# Autodesk Inventor assembly: Ecran
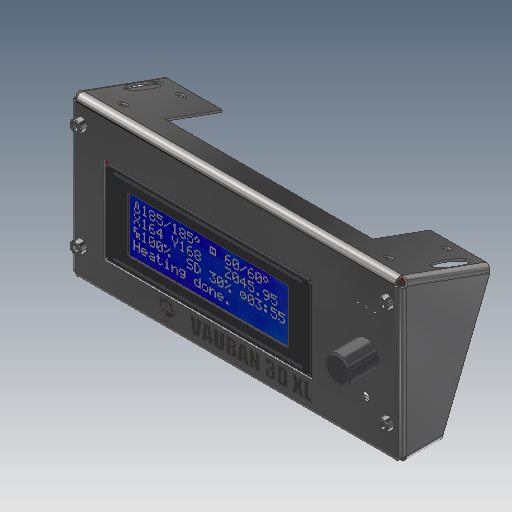
[picture p0: Inventor's stored thumbnail of the model, 512x512]
Saved by Autodesk Inventor 2017 (Build 210142000, 142)
## iProperties
Company: FABLAB Frenchmakers
Part Number: Ecran
Material: Générique
Document SubType Name: Assembly
Designer: FABLAB Frenchmakers
Project: 1420 Vauban 3D XL
Catalog Web Link: http://frenchmakers.com/
Stock Number: 1420-08-00
## Documents named in this file (6)
- W:\Professionnel\Conception FABLAB\1420-Vauban 3D XL\1420-08 Ecran\1420-08-00 Ecran.iam
- W:\Professionnel\Conception FABLAB\1420-Vauban 3D XL\1420-08 Ecran\1420-08-02 Ecran LCD.ipt
- W:\Professionnel\Conception FABLAB\1420-Vauban 3D XL\1420-90 Centre de contenu\fr-FR\ANSI B18.3.1M(1)\ANSI B18.3.1M - M3x0,5 x 20(2).ipt
- W:\Professionnel\Conception FABLAB\1420-Vauban 3D XL\1420-90 Centre de contenu\fr-FR\DIN 934\DIN 934 - M3 x 0,5.ipt
- W:\Professionnel\Conception FABLAB\1420-Vauban 3D XL\1420-08 Ecran\1420-08-01 Boitier tole.ipt
- W:\Professionnel\Conception FABLAB\1420-Vauban 3D XL\1420-08 Ecran\1420-08-03 Carte SD.ipt
## Components (19 placed, 5 different names)
1. 1420-08-02 Ecran LCD:1 — Placage:13, Placage:16, Placage:17, Placage:21, Placage:22, Placage:23, Logement:3, Logement:5, Logement:8, Logement:9, Affleurement:11
2. 1420-08-01 Boitier tole:1 — Placage:14, Affleurement:10, Placage:15, Placage:16, Placage:17, Logement:1, Placage:18, Placage:19, Placage:20, Logement:2, Logement:4, Logement:6, Logement:7, Affleurement:11
3. Vis à tête percée - Métrique M3x0,5 x 20:1 — Affleurement:4, Placage:11, Placage:19
4. Vis à tête percée - Métrique M3x0,5 x 20:2 — Affleurement:4, Affleurement:5, Placage:9, Placage:18
5. Vis à tête percée - Métrique M3x0,5 x 20:3 — Affleurement:5, Affleurement:6, Placage:10, Logement:1
6. Vis à tête percée - Métrique M3x0,5 x 20:4 — Affleurement:6, Placage:12, Placage:20
7. DIN 934 - Remplacé par DIN EN 24032/28673/28674 M3:1 — Affleurement:7, Affleurement:8, Placage:10, Placage:13
8. DIN 934 - Remplacé par DIN EN 24032/28673/28674 M3:2 — Affleurement:8, Affleurement:9, Placage:11
9. DIN 934 - Remplacé par DIN EN 24032/28673/28674 M3:3 — Affleurement:9, Placage:12
10. DIN 934 - Remplacé par DIN EN 24032/28673/28674 M3:4 — Affleurement:7, Placage:9
11. 1420-08-03 Carte SD:1 — Placage:21, Placage:22, Placage:23
12. DIN 934 - Remplacé par DIN EN 24032/28673/28674 M3:5 — Logement:3
13. DIN 934 - Remplacé par DIN EN 24032/28673/28674 M3:6 — Logement:2
14. DIN 934 - Remplacé par DIN EN 24032/28673/28674 M3:7 — Logement:5
15. DIN 934 - Remplacé par DIN EN 24032/28673/28674 M3:8 — Logement:4
16. DIN 934 - Remplacé par DIN EN 24032/28673/28674 M3:9 — Logement:9
17. DIN 934 - Remplacé par DIN EN 24032/28673/28674 M3:10 — Logement:8
18. DIN 934 - Remplacé par DIN EN 24032/28673/28674 M3:11 — Logement:7
19. DIN 934 - Remplacé par DIN EN 24032/28673/28674 M3:12 — Logement:6
## Relationships (32: Mate 15, Insert 9, Flush 8)
- Affleurement:4 [Flush]: Vis à tête percée - Métrique M3x0,5 x 20:1 ↔ Vis à tête percée - Métrique M3x0,5 x 20:2
- Affleurement:5 [Flush]: Vis à tête percée - Métrique M3x0,5 x 20:2 ↔ Vis à tête percée - Métrique M3x0,5 x 20:3
- Affleurement:6 [Flush]: Vis à tête percée - Métrique M3x0,5 x 20:3 ↔ Vis à tête percée - Métrique M3x0,5 x 20:4
- Affleurement:7 [Flush]: DIN 934 - Remplacé par DIN EN 24032/28673/28674 M3:1 ↔ DIN 934 - Remplacé par DIN EN 24032/28673/28674 M3:4
- Affleurement:8 [Flush]: DIN 934 - Remplacé par DIN EN 24032/28673/28674 M3:1 ↔ DIN 934 - Remplacé par DIN EN 24032/28673/28674 M3:2
- Affleurement:9 [Flush]: DIN 934 - Remplacé par DIN EN 24032/28673/28674 M3:2 ↔ DIN 934 - Remplacé par DIN EN 24032/28673/28674 M3:3
- Placage:9 [Mate]: Vis à tête percée - Métrique M3x0,5 x 20:2 ↔ DIN 934 - Remplacé par DIN EN 24032/28673/28674 M3:4
- Placage:10 [Mate]: Vis à tête percée - Métrique M3x0,5 x 20:3 ↔ DIN 934 - Remplacé par DIN EN 24032/28673/28674 M3:1
- Placage:11 [Mate]: Vis à tête percée - Métrique M3x0,5 x 20:1 ↔ DIN 934 - Remplacé par DIN EN 24032/28673/28674 M3:2
- Placage:12 [Mate]: Vis à tête percée - Métrique M3x0,5 x 20:4 ↔ DIN 934 - Remplacé par DIN EN 24032/28673/28674 M3:3
- Placage:13 [Mate]: 1420-08-02 Ecran LCD:1 ↔ DIN 934 - Remplacé par DIN EN 24032/28673/28674 M3:1
- Placage:14 [Mate]: 1420-08-01 Boitier tole:1
- Affleurement:10 [Flush]: 1420-08-01 Boitier tole:1
- Placage:15 [Mate]: 1420-08-01 Boitier tole:1
- Placage:16 [Mate]: 1420-08-02 Ecran LCD:1 ↔ 1420-08-01 Boitier tole:1
- Placage:17 [Mate]: 1420-08-02 Ecran LCD:1 ↔ 1420-08-01 Boitier tole:1
- Logement:1 [Insert]: 1420-08-01 Boitier tole:1 ↔ Vis à tête percée - Métrique M3x0,5 x 20:3
- Placage:18 [Mate]: 1420-08-01 Boitier tole:1 ↔ Vis à tête percée - Métrique M3x0,5 x 20:2
- Placage:19 [Mate]: 1420-08-01 Boitier tole:1 ↔ Vis à tête percée - Métrique M3x0,5 x 20:1
- Placage:20 [Mate]: 1420-08-01 Boitier tole:1 ↔ Vis à tête percée - Métrique M3x0,5 x 20:4
- Placage:21 [Mate]: 1420-08-02 Ecran LCD:1 ↔ 1420-08-03 Carte SD:1
- Placage:22 [Mate]: 1420-08-02 Ecran LCD:1 ↔ 1420-08-03 Carte SD:1
- Placage:23 [Mate]: 1420-08-02 Ecran LCD:1 ↔ 1420-08-03 Carte SD:1
- Logement:2 [Insert]: 1420-08-01 Boitier tole:1 ↔ DIN 934 - Remplacé par DIN EN 24032/28673/28674 M3:6
- Logement:3 [Insert]: 1420-08-02 Ecran LCD:1 ↔ DIN 934 - Remplacé par DIN EN 24032/28673/28674 M3:5
- Logement:4 [Insert]: 1420-08-01 Boitier tole:1 ↔ DIN 934 - Remplacé par DIN EN 24032/28673/28674 M3:8
- Logement:5 [Insert]: 1420-08-02 Ecran LCD:1 ↔ DIN 934 - Remplacé par DIN EN 24032/28673/28674 M3:7
- Logement:6 [Insert]: 1420-08-01 Boitier tole:1 ↔ DIN 934 - Remplacé par DIN EN 24032/28673/28674 M3:12
- Logement:7 [Insert]: 1420-08-01 Boitier tole:1 ↔ DIN 934 - Remplacé par DIN EN 24032/28673/28674 M3:11
- Logement:8 [Insert]: 1420-08-02 Ecran LCD:1 ↔ DIN 934 - Remplacé par DIN EN 24032/28673/28674 M3:10
- Logement:9 [Insert]: 1420-08-02 Ecran LCD:1 ↔ DIN 934 - Remplacé par DIN EN 24032/28673/28674 M3:9
- Affleurement:11 [Flush]: 1420-08-02 Ecran LCD:1 ↔ 1420-08-01 Boitier tole:1
